# Autodesk Inventor assembly: 홀간 거리 확인-1
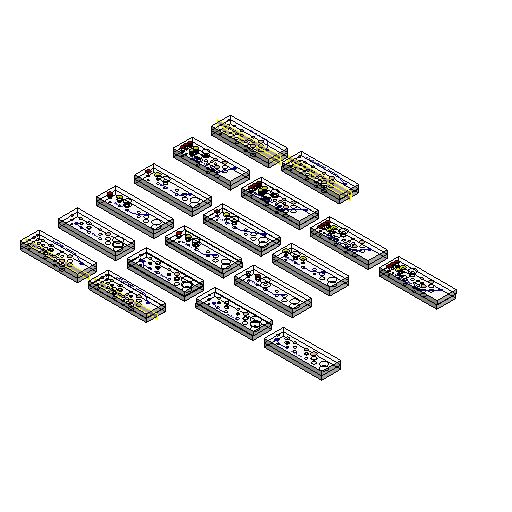
[picture p0: Inventor's stored thumbnail of the model, 512x512]
Saved by Autodesk Inventor 2026.1 (Build 301233000, 233)
## iProperties
Category: Title of a parent object over this object
Company: Customer
RuleStatus: InUse
Created: 2025-12-05
Part Number: 홀간 거리 확인-1
Project: Project Number
Checked By: Designed
Engr Approved By: Checked
User Status: set
Material: SS400
Description: Description
Document SubType Name: Assembly
Mfg Approved By: Approved
Designer: suhyun-yoon
Stock Number: Stock Number
Deteil Description: Detail Description
Title: This Unit Title
Subject: Project Name
Author: suhyun-yoon
Revision Number: A
## Documents named in this file (13)
- D:\V\Designs\TRAIN\윤수현(ilogic test)\홀간 거리 확인-1.iam
- D:\V\Designs\TRAIN\윤수현(ilogic test)\홀간 거리 확인 파트-1.ipt
- D:\V\Designs\TRAIN\윤수현(ilogic test)\홀간 거리 확인 파트-2.ipt
- D:\V\Designs\TRAIN\윤수현(ilogic test)\홀간 거리 확인 파트-3.ipt
- D:\V\Designs\TRAIN\윤수현(ilogic test)\홀간 거리 확인 파트-4.ipt
- D:\V\Designs\TRAIN\윤수현(ilogic test)\홀간 거리 확인 파트-6.ipt
- D:\V\Designs\TRAIN\윤수현(ilogic test)\홀간 거리 확인 파트-7.ipt
- D:\V\Designs\TRAIN\윤수현(ilogic test)\홀간 거리 확인 파트-8.ipt
- D:\V\Designs\TRAIN\윤수현(ilogic test)\홀간 거리 확인 파트-9.ipt
- D:\V\Designs\TRAIN\윤수현(ilogic test)\홀간 거리 확인 파트-10.ipt
- D:\V\Designs\TRAIN\윤수현(ilogic test)\홀간 거리 확인 파트-10_CPY.ipt
- D:\V\Designs\TRAIN\윤수현(ilogic test)\홀간 거리 확인 파트-12.ipt
- D:\V\Designs\TRAIN\윤수현(ilogic test)\홀간 거리 확인 파트-13.ipt
## Components (36 placed, 12 different names)
1. 홀간 거리 확인 파트-1:1 — Mate:1, Flush:1, Flush:2, Mate:7, Flush:13, Flush:14, Flush:19, Flush:27
2. 홀간 거리 확인 파트-1:2 — Mate:6, Mate:7, Flush:13, Flush:14, Mate:9, Flush:17, Flush:18
3. 홀간 거리 확인 파트-1:3 — Mate:9, Flush:17, Flush:18
4. 홀간 거리 확인 파트-2:1 — Mate:1, Flush:1, Flush:2, Flush:24, Mate:11, Flush:45, Mate:21, Flush:46
5. 홀간 거리 확인 파트-2:3 — Mate:6
6. 홀간 거리 확인 파트-2:4 — Mate:18, Flush:38, Flush:39
7. 홀간 거리 확인 파트-2:5 — Flush:24, Mate:11, Flush:25, Flush:26, Mate:12, Flush:57, Flush:58, Mate:27
8. 홀간 거리 확인 파트-2:6 — Mate:16, Flush:35, Flush:44
9. 홀간 거리 확인 파트-2:7 — Mate:16, Flush:35, Mate:20, Flush:42, Flush:43, Flush:44
10. 홀간 거리 확인 파트-2:8 — Mate:18, Flush:38, Flush:39, Mate:19, Flush:40, Flush:41
11. 홀간 거리 확인 파트-3:1 — Flush:19, Flush:65, Flush:68, Mate:31, Mate:34, Flush:71, Flush:72, Flush:75, Mate:36, Flush:80, Flush:81, Mate:39
12. 홀간 거리 확인 파트-4:2 — Flush:80, Flush:81, Mate:39, Mate:41, Flush:84, Flush:85
13. 홀간 거리 확인 파트-6:1 — Flush:25, Flush:26, Mate:12, Flush:27, Flush:30, Flush:31, Mate:14
14. 홀간 거리 확인 파트-6:2 — Flush:30, Flush:31, Mate:14
15. 홀간 거리 확인 파트-7:1 — Mate:19, Flush:40, Flush:41
16. 홀간 거리 확인 파트-8:1 — Mate:20, Flush:42, Flush:43
17. 홀간 거리 확인 파트-4:3 — Flush:45, Mate:21, Flush:46, Mate:22, Flush:47, Flush:48, Mate:23, Flush:49, Flush:50
18. 홀간 거리 확인 파트-4:4 — Mate:22, Flush:47, Flush:48, Mate:24, Flush:51, Flush:52
19. 홀간 거리 확인 파트-9:1 — Mate:23, Flush:49, Flush:50
20. 홀간 거리 확인 파트-9:2 — Mate:24, Flush:51, Flush:52
21. 홀간 거리 확인 파트-2:9 — Flush:55, Flush:56, Mate:26, Flush:57, Flush:58, Mate:27, Mate:28, Flush:59, Flush:60, Flush:75, Mate:36
22. 홀간 거리 확인 파트-2:10 — Flush:55, Flush:56, Mate:26, Mate:30, Flush:63, Flush:64
23. 홀간 거리 확인 파트-2:11 — Mate:29, Flush:61, Flush:62
24. 홀간 거리 확인 파트-10:1 — Mate:28, Flush:59, Flush:60
25. 홀간 거리 확인 파트-11:1 — Mate:29, Flush:61, Flush:62
26. 홀간 거리 확인 파트-10:2 — Mate:30, Flush:63, Flush:64
27. 홀간 거리 확인 파트-3:2 — Flush:65, Flush:66, Flush:68, Flush:69, Mate:31, Mate:32, Mate:35, Flush:73, Flush:74
28. 홀간 거리 확인 파트-3:3 — Flush:66, Flush:67, Flush:69, Flush:70, Mate:32, Mate:33, Mate:37, Flush:76, Flush:77
29. 홀간 거리 확인 파트-3:4 — Flush:67, Flush:70, Mate:33, Mate:38, Flush:78, Flush:79
30. 홀간 거리 확인 파트-12:1 — Mate:34, Flush:71, Flush:72
31. 홀간 거리 확인 파트-13:1 — Mate:37, Flush:76, Flush:77
32. 홀간 거리 확인 파트-12:2 — Mate:35, Flush:73, Flush:74
33. 홀간 거리 확인 파트-13:2 — Mate:38, Flush:78, Flush:79
34. 홀간 거리 확인 파트-4:5 — Mate:42, Flush:86, Flush:87
35. 홀간 거리 확인 파트-4:6 — Mate:41, Flush:84, Flush:85
36. 홀간 거리 확인 파트-4:7 — Mate:42, Flush:86, Flush:87
## Relationships (102: Flush 68, Mate 34)
- Mate:1: 홀간 거리 확인 파트-1:1 ↔ 홀간 거리 확인 파트-2:1
- Flush:1: 홀간 거리 확인 파트-1:1 ↔ 홀간 거리 확인 파트-2:1
- Flush:2: 홀간 거리 확인 파트-1:1 ↔ 홀간 거리 확인 파트-2:1
- Mate:6 (2 mm): 홀간 거리 확인 파트-1:2 ↔ 홀간 거리 확인 파트-2:3
- [Flush]: 홀간 거리 확인 파트-1:2 ↔ 홀간 거리 확인 파트-2:3
- [Flush]: 홀간 거리 확인 파트-1:2 ↔ 홀간 거리 확인 파트-2:3
- Mate:7 (30 mm): 홀간 거리 확인 파트-1:1 ↔ 홀간 거리 확인 파트-1:2
- Flush:13: 홀간 거리 확인 파트-1:1 ↔ 홀간 거리 확인 파트-1:2
- Flush:14: 홀간 거리 확인 파트-1:1 ↔ 홀간 거리 확인 파트-1:2
- [Mate]: 홀간 거리 확인 파트-1:3 ↔ 홀간 거리 확인 파트-2:4
- [Flush] (1.5 mm): 홀간 거리 확인 파트-1:3 ↔ 홀간 거리 확인 파트-2:4
- [Flush]: 홀간 거리 확인 파트-1:3 ↔ 홀간 거리 확인 파트-2:4
- Mate:9 (30 mm): 홀간 거리 확인 파트-1:2 ↔ 홀간 거리 확인 파트-1:3
- Flush:17: 홀간 거리 확인 파트-1:2 ↔ 홀간 거리 확인 파트-1:3
- Flush:18: 홀간 거리 확인 파트-1:2 ↔ 홀간 거리 확인 파트-1:3
- Flush:19: 홀간 거리 확인 파트-1:1 ↔ 홀간 거리 확인 파트-3:1
- Flush:24: 홀간 거리 확인 파트-2:1 ↔ 홀간 거리 확인 파트-2:5
- Mate:11 (50 mm): 홀간 거리 확인 파트-2:1 ↔ 홀간 거리 확인 파트-2:5
- Flush:25: 홀간 거리 확인 파트-2:5 ↔ 홀간 거리 확인 파트-6:1
- Flush:26: 홀간 거리 확인 파트-2:5 ↔ 홀간 거리 확인 파트-6:1
- Mate:12: 홀간 거리 확인 파트-2:5 ↔ 홀간 거리 확인 파트-6:1
- Flush:27: 홀간 거리 확인 파트-1:1 ↔ 홀간 거리 확인 파트-6:1
- [Flush] (1.3 mm): 홀간 거리 확인 파트-2:6 ↔ 홀간 거리 확인 파트-6:2
- [Flush]: 홀간 거리 확인 파트-2:6 ↔ 홀간 거리 확인 파트-6:2
- [Mate]: 홀간 거리 확인 파트-2:6 ↔ 홀간 거리 확인 파트-6:2
- Flush:30: 홀간 거리 확인 파트-6:1 ↔ 홀간 거리 확인 파트-6:2
- Flush:31: 홀간 거리 확인 파트-6:1 ↔ 홀간 거리 확인 파트-6:2
- Mate:14 (30 mm): 홀간 거리 확인 파트-6:1 ↔ 홀간 거리 확인 파트-6:2
- Mate:16 (30 mm): 홀간 거리 확인 파트-2:6 ↔ 홀간 거리 확인 파트-2:7
- Flush:35: 홀간 거리 확인 파트-2:6 ↔ 홀간 거리 확인 파트-2:7
- Mate:18 (30 mm): 홀간 거리 확인 파트-2:4 ↔ 홀간 거리 확인 파트-2:8
- Flush:38: 홀간 거리 확인 파트-2:4 ↔ 홀간 거리 확인 파트-2:8
- Flush:39: 홀간 거리 확인 파트-2:4 ↔ 홀간 거리 확인 파트-2:8
- Mate:19: 홀간 거리 확인 파트-2:8 ↔ 홀간 거리 확인 파트-7:1
- Flush:40: 홀간 거리 확인 파트-2:8 ↔ 홀간 거리 확인 파트-7:1
- Flush:41: 홀간 거리 확인 파트-2:8 ↔ 홀간 거리 확인 파트-7:1
- Mate:20: 홀간 거리 확인 파트-2:7 ↔ 홀간 거리 확인 파트-8:1
- Flush:42: 홀간 거리 확인 파트-2:7 ↔ 홀간 거리 확인 파트-8:1
- Flush:43: 홀간 거리 확인 파트-2:7 ↔ 홀간 거리 확인 파트-8:1
- Flush:44: 홀간 거리 확인 파트-2:6 ↔ 홀간 거리 확인 파트-2:7
- Flush:45: 홀간 거리 확인 파트-2:1 ↔ 홀간 거리 확인 파트-4:3
- Mate:21 (50 mm): 홀간 거리 확인 파트-2:1 ↔ 홀간 거리 확인 파트-4:3
- Flush:46: 홀간 거리 확인 파트-2:1 ↔ 홀간 거리 확인 파트-4:3
- Mate:22 (30 mm): 홀간 거리 확인 파트-4:3 ↔ 홀간 거리 확인 파트-4:4
- Flush:47: 홀간 거리 확인 파트-4:3 ↔ 홀간 거리 확인 파트-4:4
- Flush:48: 홀간 거리 확인 파트-4:3 ↔ 홀간 거리 확인 파트-4:4
- Mate:23: 홀간 거리 확인 파트-4:3 ↔ 홀간 거리 확인 파트-9:1
- Flush:49: 홀간 거리 확인 파트-4:3 ↔ 홀간 거리 확인 파트-9:1
- Flush:50: 홀간 거리 확인 파트-4:3 ↔ 홀간 거리 확인 파트-9:1
- Mate:24: 홀간 거리 확인 파트-4:4 ↔ 홀간 거리 확인 파트-9:2
- Flush:51 (0.7 mm): 홀간 거리 확인 파트-4:4 ↔ 홀간 거리 확인 파트-9:2
- Flush:52 (0.7 mm): 홀간 거리 확인 파트-4:4 ↔ 홀간 거리 확인 파트-9:2
- [Mate] (30 mm): 홀간 거리 확인 파트-2:10 ↔ 홀간 거리 확인 파트-2:11
- [Flush]: 홀간 거리 확인 파트-2:10 ↔ 홀간 거리 확인 파트-2:11
- [Flush]: 홀간 거리 확인 파트-2:10 ↔ 홀간 거리 확인 파트-2:11
- Flush:55: 홀간 거리 확인 파트-2:9 ↔ 홀간 거리 확인 파트-2:10
- Flush:56: 홀간 거리 확인 파트-2:9 ↔ 홀간 거리 확인 파트-2:10
- Mate:26 (30 mm): 홀간 거리 확인 파트-2:9 ↔ 홀간 거리 확인 파트-2:10
- Flush:57: 홀간 거리 확인 파트-2:5 ↔ 홀간 거리 확인 파트-2:9
- Flush:58: 홀간 거리 확인 파트-2:5 ↔ 홀간 거리 확인 파트-2:9
- Mate:27 (50 mm): 홀간 거리 확인 파트-2:5 ↔ 홀간 거리 확인 파트-2:9
- Mate:28: 홀간 거리 확인 파트-2:9 ↔ 홀간 거리 확인 파트-10:1
- Flush:59: 홀간 거리 확인 파트-2:9 ↔ 홀간 거리 확인 파트-10:1
- Flush:60: 홀간 거리 확인 파트-2:9 ↔ 홀간 거리 확인 파트-10:1
- Mate:29: 홀간 거리 확인 파트-2:11 ↔ 홀간 거리 확인 파트-11:1
- Flush:61: 홀간 거리 확인 파트-2:11 ↔ 홀간 거리 확인 파트-11:1
- Flush:62: 홀간 거리 확인 파트-2:11 ↔ 홀간 거리 확인 파트-11:1
- Mate:30: 홀간 거리 확인 파트-2:10 ↔ 홀간 거리 확인 파트-10:2
- Flush:63 (0.6 mm): 홀간 거리 확인 파트-2:10 ↔ 홀간 거리 확인 파트-10:2
- Flush:64 (0.6 mm): 홀간 거리 확인 파트-2:10 ↔ 홀간 거리 확인 파트-10:2
- Flush:65: 홀간 거리 확인 파트-3:1 ↔ 홀간 거리 확인 파트-3:2
- Flush:66: 홀간 거리 확인 파트-3:2 ↔ 홀간 거리 확인 파트-3:3
- Flush:67: 홀간 거리 확인 파트-3:3 ↔ 홀간 거리 확인 파트-3:4
- Flush:68: 홀간 거리 확인 파트-3:1 ↔ 홀간 거리 확인 파트-3:2
- Flush:69: 홀간 거리 확인 파트-3:2 ↔ 홀간 거리 확인 파트-3:3
- Flush:70: 홀간 거리 확인 파트-3:3 ↔ 홀간 거리 확인 파트-3:4
- Mate:31 (30 mm): 홀간 거리 확인 파트-3:1 ↔ 홀간 거리 확인 파트-3:2
- Mate:32 (30 mm): 홀간 거리 확인 파트-3:2 ↔ 홀간 거리 확인 파트-3:3
- Mate:33 (30 mm): 홀간 거리 확인 파트-3:3 ↔ 홀간 거리 확인 파트-3:4
- Mate:34: 홀간 거리 확인 파트-3:1 ↔ 홀간 거리 확인 파트-12:1
- Flush:71: 홀간 거리 확인 파트-3:1 ↔ 홀간 거리 확인 파트-12:1
- Flush:72: 홀간 거리 확인 파트-3:1 ↔ 홀간 거리 확인 파트-12:1
- Mate:35: 홀간 거리 확인 파트-3:2 ↔ 홀간 거리 확인 파트-12:2
- Flush:73 (0.5 mm): 홀간 거리 확인 파트-3:2 ↔ 홀간 거리 확인 파트-12:2
- Flush:74 (0.5 mm): 홀간 거리 확인 파트-3:2 ↔ 홀간 거리 확인 파트-12:2
- Flush:75: 홀간 거리 확인 파트-3:1 ↔ 홀간 거리 확인 파트-2:9
- Mate:36 (50 mm): 홀간 거리 확인 파트-3:1 ↔ 홀간 거리 확인 파트-2:9
- Mate:37: 홀간 거리 확인 파트-3:3 ↔ 홀간 거리 확인 파트-13:1
- Flush:76: 홀간 거리 확인 파트-3:3 ↔ 홀간 거리 확인 파트-13:1
- Flush:77: 홀간 거리 확인 파트-3:3 ↔ 홀간 거리 확인 파트-13:1
- Mate:38: 홀간 거리 확인 파트-3:4 ↔ 홀간 거리 확인 파트-13:2
- Flush:78: 홀간 거리 확인 파트-3:4 ↔ 홀간 거리 확인 파트-13:2
- Flush:79 (0.5 mm): 홀간 거리 확인 파트-3:4 ↔ 홀간 거리 확인 파트-13:2
- Flush:80: 홀간 거리 확인 파트-3:1 ↔ 홀간 거리 확인 파트-4:2
- Flush:81: 홀간 거리 확인 파트-3:1 ↔ 홀간 거리 확인 파트-4:2
- Mate:39 (50 mm): 홀간 거리 확인 파트-3:1 ↔ 홀간 거리 확인 파트-4:2
- Mate:41: 홀간 거리 확인 파트-4:2 ↔ 홀간 거리 확인 파트-4:6
- Flush:84: 홀간 거리 확인 파트-4:2 ↔ 홀간 거리 확인 파트-4:6
- Flush:85: 홀간 거리 확인 파트-4:2 ↔ 홀간 거리 확인 파트-4:6
- Mate:42: 홀간 거리 확인 파트-4:5 ↔ 홀간 거리 확인 파트-4:7
- Flush:86: 홀간 거리 확인 파트-4:5 ↔ 홀간 거리 확인 파트-4:7
- Flush:87 (1 mm): 홀간 거리 확인 파트-4:5 ↔ 홀간 거리 확인 파트-4:7
## Named parameters: d1782_d1740 = 2 mm, d1783_d1741 = 0 mm, d1784_d1742 = 0 mm, d1788_d1740 = 0 mm, d1789_d1741 = 1.5 mm, d1790_d1742 = 0 mm, d1817_d1813 = 1.3 mm, d1818_d1814 = 0 mm, d1819_d1815 = 0 mm, d1866_d1847 = 0 mm, d1867_d1831 = 30 mm, d1868_d1832 = 0 mm
